# Autodesk Inventor assembly: Assembly1
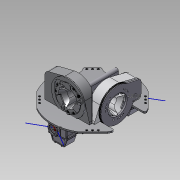
[picture p0: Inventor's stored thumbnail of the model, 180x180]
Saved by Autodesk Inventor 2011 (Build 150239000, 239)
## iProperties
Created: 2011-03-18
Part Number: Assembly1
Document SubType Name: Assembly
Designer: casey
Author: casey
## Documents named in this file (8)
- C:\Users\Casey\Documents\My Dropbox\RockSAT-X 2011 RexSAT\capsule-launcher.design\Full assembly.iam
- C:\Users\Casey\Documents\My Dropbox\RockSAT-X 2011 RexSAT\capsule-launcher.design\Deck.ipt
- C:\Users\Casey\Documents\My Dropbox\RockSAT-X 2011 RexSAT\capsule-launcher.design\Launcher\launcher.mainAssembly.iam
- C:\Users\Casey\Documents\My Dropbox\RockSAT-X 2011 RexSAT\capsule-launcher.design\Camera\Camera.assembly.iam
- C:\Users\Casey\Documents\My Dropbox\RockSAT-X 2011 RexSAT\capsule-launcher.design\Launcher\Pusher.iam
- C:\Users\Casey\Documents\My Dropbox\RockSAT-X 2011 RexSAT\capsule-launcher.design\Launcher\launcher.mainAssembly2.iam
- C:\Users\Casey\Documents\My Dropbox\RockSAT-X 2011 RexSAT\capsule-launcher.design\Launcher\Pusher2.iam
- C:\Users\Casey\Documents\My Dropbox\RockSAT-X 2011 RexSAT\capsule-launcher.design\Electronics Box\Base.Box.Base.ipt
## Components (8 placed, 7 different names)
1. Deck:1 — Mate:9, Mate:12, Mate:13, Mate:14, Mate:15, Mate:16, Mate:19, Mate:22, Mate:29
2. Camera.assembly:1 [sub-assembly] — Mate:9
3. Camera.assembly:3 [sub-assembly] — Mate:12
4. launcher.mainAssembly:1 [sub-assembly] — Mate:13, Mate:14, Mate:15, Mate:16
5. Pusher:1 [sub-assembly] — Mate:19, Mate:31
6. launcher.mainAssembly2:1 [sub-assembly] — Mate:22, Angle:1
7. Pusher2:1 [sub-assembly] — Mate:29, Flush:1, Mate:31
8. Base.Box.Base:1
## Relationships (12: Mate 10, Flush 1, Angle 1)
- Mate:9: Deck:1 ↔ Camera.assembly:1
- Mate:12: Deck:1 ↔ Camera.assembly:3
- Mate:13: Deck:1 ↔ launcher.mainAssembly:1
- Mate:14: Deck:1 ↔ launcher.mainAssembly:1
- Mate:15: Deck:1 ↔ launcher.mainAssembly:1
- Mate:16: Deck:1 ↔ launcher.mainAssembly:1
- Mate:19: Deck:1 ↔ Pusher:1
- Mate:22: Deck:1 ↔ launcher.mainAssembly2:1
- Mate:29: Deck:1 ↔ Pusher2:1
- Flush:1: Pusher2:1
- Angle:1 (0 deg): launcher.mainAssembly2:1
- Mate:31: Pusher:1 ↔ Pusher2:1
